# Autodesk Inventor assembly: ASM_Testing
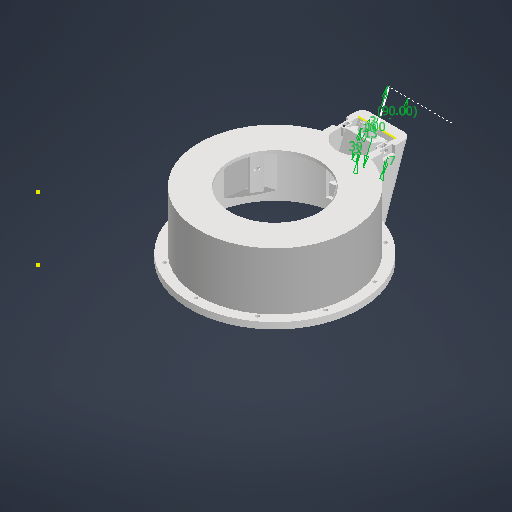
[picture p0: Inventor's stored thumbnail of the model, 512x512]
Saved by Autodesk Inventor 2026 (Build 300175000, 175)
## iProperties
Created: 2025-09-29
Part Number: ASM_Testing
Document SubType Name: Assembly
Designer: Charl
Author: Charl
## Documents named in this file (3)
- C:\School\Research\Inventor\v0.4\ASM_Testing.iam
- C:\School\Research\Inventor\v0.4\Cylinder_Housing_Event.ipt
- C:\School\Research\Inventor\v0.3\Camera\Triton2_asm.iam
## Components (2 placed, 2 different names)
1. Cylinder_Housing_Event:1 — Mate:1, Mate:2
2. Triton2_asm:1 [sub-assembly] — Mate:1, Mate:2
## Relationships (2: Mate 2)
- Mate:1: Cylinder_Housing_Event:1 ↔ Triton2_asm:1
- Mate:2: Cylinder_Housing_Event:1 ↔ Triton2_asm:1
